# Autodesk Inventor assembly: Assembly1
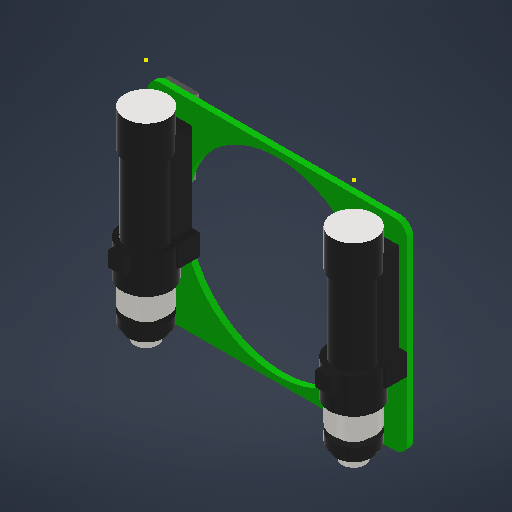
[picture p0: Inventor's stored thumbnail of the model, 512x512]
Saved by Autodesk Inventor 2026.1 (Build 301233000, 233)
## iProperties
Created: 2025-11-06
Part Number: Assembly1
Document SubType Name: Assembly
Designer: SPEL
Author: SPEL
## Documents named in this file (3)
- C:\Users\SPEL\Desktop\SPEL\Femto\Assembly1.iam
- C:\Users\SPEL\Desktop\SPEL\Femto\PCB.ipt
- C:\Users\SPEL\Desktop\SPEL\Femto\injector femto.ipt
## Components (3 placed, 2 different names)
1. PCB:1 — Flush:1, Mate:1, Flush:2, Flush:3, Mate:2, Flush:4
2. injector femto:1 — Flush:1, Mate:1, Flush:2
3. injector femto:2 — Flush:3, Mate:2, Flush:4
## Relationships (6: Flush 4, Mate 2)
- Flush:1: PCB:1 ↔ injector femto:1
- Mate:1: PCB:1 ↔ injector femto:1
- Flush:2: PCB:1 ↔ injector femto:1
- Flush:3: PCB:1 ↔ injector femto:2
- Mate:2: PCB:1 ↔ injector femto:2
- Flush:4: PCB:1 ↔ injector femto:2
